# Autodesk Inventor assembly: ensemble
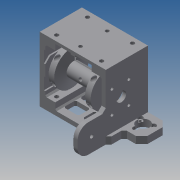
[picture p0: Inventor's stored thumbnail of the model, 180x180]
Saved by Autodesk Inventor 2019 (Build 230136000, 136)
## iProperties
Created: 2020-07-07
Part Number: ensemble
Material: Générique
Document SubType Name: Assembly
Designer: Theo
Author: Theo
## Documents named in this file (7)
- D:\dev\projects\trape_poules\ensemble.iam
- D:\dev\projects\trape_poules\attache_moteur.ipt
- D:\dev\projects\trape_poules\cloison_reducteur.ipt
- D:\dev\projects\trape_poules\cloison_exterieur.ipt
- D:\dev\projects\trape_poules\demi_tambour.ipt
- D:\dev\projects\trape_poules\demi_tambour_ecrous.ipt
- D:\dev\projects\trape_poules\attache_exterieur.ipt
## Components (6 placed, 6 different names)
1. attache_moteur:1 — Placage:1, Logement:1, Logement:2, Placage:2, Logement:3, Logement:4
2. cloison_reducteur:1 — Placage:1, Logement:1, Logement:2, Placage:3
3. cloison_exterieur:1 — Placage:2, Logement:3, Logement:4, Placage:5, Affleurement:1, Affleurement:2
4. demi_tambour:1 — Placage:3, Placage:4
5. demi_tambour_ecrous:1 — Placage:4
6. attache_exterieur:1 — Placage:5, Affleurement:1, Affleurement:2
## Relationships (11: Mate 5, Insert 4, Flush 2)
- Placage:1 [Mate]: attache_moteur:1 ↔ cloison_reducteur:1
- Logement:1 [Insert]: attache_moteur:1 ↔ cloison_reducteur:1
- Logement:2 [Insert]: attache_moteur:1 ↔ cloison_reducteur:1
- Placage:2 [Mate]: attache_moteur:1 ↔ cloison_exterieur:1
- Logement:3 [Insert]: attache_moteur:1 ↔ cloison_exterieur:1
- Logement:4 [Insert]: attache_moteur:1 ↔ cloison_exterieur:1
- Placage:3 [Mate]: cloison_reducteur:1 ↔ demi_tambour:1
- Placage:4 [Mate]: demi_tambour:1 ↔ demi_tambour_ecrous:1
- Placage:5 [Mate]: cloison_exterieur:1 ↔ attache_exterieur:1
- Affleurement:1 [Flush]: cloison_exterieur:1 ↔ attache_exterieur:1
- Affleurement:2 [Flush]: cloison_exterieur:1 ↔ attache_exterieur:1
